# Autodesk Inventor assembly: A2017_T5_01
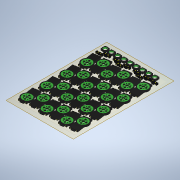
[picture p0: Inventor's stored thumbnail of the model, 180x180]
Saved by Autodesk Inventor 2022 (Build 260153000, 153)
## iProperties
Created: 2022-09-28
Part Number: A2017_T5_01
Document SubType Name: Assembly
Designer: Masato
Author: Masato
## Documents named in this file (5)
- C:\Users\6343y\ドキュメント\Inventor\SUSTAINA-OP\Cam\A2017_T5\A2017_T5_01.iam
- C:\Users\6343y\ドキュメント\Inventor\SUSTAINA-OP\Cam\DisposableBoard.ipt
- C:\Users\6343y\ドキュメント\Inventor\SUSTAINA-OP\LowerBody\Leg_joint\Leg_joint_yaw_frame.ipt
- C:\Users\6343y\ドキュメント\Inventor\SUSTAINA-OP\LowerBody\Knee\Knee_clamp.ipt
- C:\Users\6343y\ドキュメント\Inventor\SUSTAINA-OP\LowerBody\Foot\Foot_root_block.ipt
## Components (43 placed, 4 different names)
1. DisposableBoard:1 — フラッシュ:1, フラッシュ:2, フラッシュ:3, フラッシュ:4, 正接:1, メイト:3, メイト:4, 正接:12, 正接:13, 正接:14, フラッシュ:5
2. Foot_root_block:11 — メイト:13, メイト:14, フラッシュ:6
3. Knee_clamp:2 — メイト:5, 正接:12, 正接:13, 正接:14
4. Knee_clamp:3 — 正接:15
5. Knee_clamp:4
6. Knee_clamp:5
7. Knee_clamp:6
8. Knee_clamp:7
9. Knee_clamp:8
10. Knee_clamp:9
11. Knee_clamp:10
12. Leg_joint_yaw_frame:1 — メイト:1, 正接:1, 正接:2, メイト:3, メイト:4, 正接:3, 正接:4
13. Leg_joint_yaw_frame:2 — メイト:2, 正接:2, 正接:3, 正接:4
14. Leg_joint_yaw_frame:3
15. Leg_joint_yaw_frame:4
16. Leg_joint_yaw_frame:5
17. Leg_joint_yaw_frame:6
18. Leg_joint_yaw_frame:7
19. Leg_joint_yaw_frame:8
20. Leg_joint_yaw_frame:9
21. Leg_joint_yaw_frame:10
22. Leg_joint_yaw_frame:11
23. Leg_joint_yaw_frame:12
24. Leg_joint_yaw_frame:13
25. Leg_joint_yaw_frame:14
26. Leg_joint_yaw_frame:15
27. Leg_joint_yaw_frame:16
28. Leg_joint_yaw_frame:17
29. Leg_joint_yaw_frame:18
30. Leg_joint_yaw_frame:19
31. Leg_joint_yaw_frame:20
32. Leg_joint_yaw_frame:21
33. Leg_joint_yaw_frame:22
34. Leg_joint_yaw_frame:23
35. Leg_joint_yaw_frame:24
36. Foot_root_block:2 — メイト:7, フラッシュ:5, メイト:8, メイト:9
37. Foot_root_block:7 — メイト:11, メイト:12
38. Foot_root_block:8
39. Foot_root_block:1 — メイト:6, 正接:15, メイト:8, メイト:9
40. Foot_root_block:5
41. Foot_root_block:6 — メイト:14, フラッシュ:6
42. Foot_root_block:9 — メイト:10, メイト:11, メイト:12
43. Foot_root_block:10
## Component patterns: (9 elements, first: Knee_clamp:2), (12 elements, first: Leg_joint_yaw_frame:1 + Leg_joint_yaw_frame:2), (3 elements, first: Foot_root_block:2), (3 elements, first: Foot_root_block:1), (2 elements, first: Foot_root_block:9)
## Relationships (28: Mate 14, Tangent 8, Flush 6)
- フラッシュ:1 [Flush]: DisposableBoard:1
- フラッシュ:2 [Flush]: DisposableBoard:1
- フラッシュ:3 [Flush]: DisposableBoard:1
- フラッシュ:4 [Flush]: DisposableBoard:1
- メイト:1 [Mate]: Leg_joint_yaw_frame:1
- メイト:2 [Mate]: Leg_joint_yaw_frame:2
- 正接:1 [Tangent] (2.063 mm): DisposableBoard:1 ↔ Leg_joint_yaw_frame:1
- 正接:2 [Tangent] (2.1 mm): Leg_joint_yaw_frame:1 ↔ Leg_joint_yaw_frame:2
- メイト:3 [Mate] (-2.063 mm): DisposableBoard:1 ↔ Leg_joint_yaw_frame:1
- メイト:4 [Mate] (-2.1 mm): DisposableBoard:1 ↔ Leg_joint_yaw_frame:1
- 正接:3 [Tangent] (2.1 mm): Leg_joint_yaw_frame:1 ↔ Leg_joint_yaw_frame:2
- 正接:4 [Tangent] (2.1 mm): Leg_joint_yaw_frame:1 ↔ Leg_joint_yaw_frame:2
- メイト:5 [Mate]: Knee_clamp:2
- 正接:12 [Tangent] (2.1 mm): DisposableBoard:1 ↔ Knee_clamp:2
- メイト:6 [Mate]: Foot_root_block:1
- 正接:13 [Tangent] (2.1 mm): DisposableBoard:1 ↔ Knee_clamp:2
- 正接:14 [Tangent] (2.1 mm): DisposableBoard:1 ↔ Knee_clamp:2
- メイト:7 [Mate]: Foot_root_block:2
- フラッシュ:5 [Flush] (2.1 mm): DisposableBoard:1 ↔ Foot_root_block:2
- 正接:15 [Tangent] (2.1 mm): Knee_clamp:3 ↔ Foot_root_block:1
- メイト:8 [Mate] (2.1 mm): Foot_root_block:2 ↔ Foot_root_block:1
- メイト:9 [Mate] (2.1 mm): Foot_root_block:2 ↔ Foot_root_block:1
- メイト:10 [Mate]: Foot_root_block:9
- メイト:11 [Mate] (2.1 mm): Foot_root_block:7 ↔ Foot_root_block:9
- メイト:12 [Mate] (2.1 mm): Foot_root_block:7 ↔ Foot_root_block:9
- メイト:13 [Mate]: Foot_root_block:11
- メイト:14 [Mate] (2.1 mm): Foot_root_block:11 ↔ Foot_root_block:6
- フラッシュ:6 [Flush]: Foot_root_block:11 ↔ Foot_root_block:6
